# Autodesk Inventor assembly: 08 ASY GBK wall shield 1.3.8
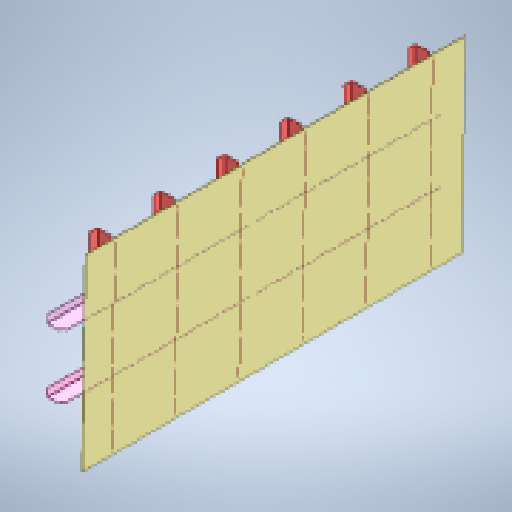
[picture p0: Inventor's stored thumbnail of the model, 512x512]
Saved by Autodesk Inventor 2026 (Build 300175000, 175)
## iProperties
Created: 2026-05-07
Part Number: 08 ASY GBK wall shield 1.3.8
Document SubType Name: Assembly
Designer: pokla
Mass: 245734 g
Surface Area: 167509 cm^2
Volume: 31303.7 cm^3
Density: 7.85 g/cm^3
Author: admin
## Documents named in this file (5)
- C:\Users\pokla\Documents\Inventor\GBK-Gubkinskiy\08 ASY GBK wall shield 1.3.8.iam
- C:\Users\pokla\Documents\Inventor\GBK-Gubkinskiy\0138 GBK shield 8.ipt
- C:\Users\pokla\Documents\Inventor\GBK-Gubkinskiy\08.2 GBK rib.ipt
- C:\Users\pokla\Documents\Inventor\GBK-Gubkinskiy\0381 GBK stringer 7.ipt
- C:\Users\pokla\Documents\Inventor\GBK-Gubkinskiy\0382 GBK stringer 8.ipt
## Components (11 placed, 4 different names)
1. 0381 GBK stringer 7:1
2. 0382 GBK stringer 8:1
3. 0382 GBK stringer 8:2
4. 0381 GBK stringer 7:2
5. 0138 GBK shield 8:1
6. 08.2 GBK rib:1
7. 08.2 GBK rib:2
8. 08.2 GBK rib:3
9. 08.2 GBK rib:4
10. 08.2 GBK rib:5
11. 08.2 GBK rib:6
## Component patterns: (6 elements, first: 08.2 GBK rib:1)
## Relationships (7: WeldJoint 4, Mate 2, Flush 1)
- [Flush] (250 mm): 0138 GBK shield 8:1 ↔ 08.2 GBK rib:1
- [Mate]: 0138 GBK shield 8:1 ↔ 08.2 GBK rib:1
- [Mate]: 0138 GBK shield 8:1 ↔ 08.2 GBK rib:1
- [WeldJoint] (4 mm): 0381 GBK stringer 7:1 ↔ 08.2 GBK rib:1
- [WeldJoint] (4 mm): 0382 GBK stringer 8:1 ↔ 08.2 GBK rib:1
- [WeldJoint]: 0381 GBK stringer 7:1 ↔ 0381 GBK stringer 7:2
- [WeldJoint]: 0382 GBK stringer 8:1 ↔ 0382 GBK stringer 8:2
